# Autodesk Inventor assembly: Baugruppe1
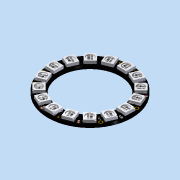
[picture p0: Inventor's stored thumbnail of the model, 180x180]
Saved by Autodesk Inventor 2015 (Build 190159000, 159)
## iProperties
Created: 2015-06-28
Part Number: Baugruppe1
Document SubType Name: Assembly
Designer: M45t3r 0f H4rdc0r3
Author: M45t3r 0f H4rdc0r3
## Documents named in this file (5)
- D:\3D Konstruktion\Neopixelring16x\Dokumentation\Baugruppe1.iam
- D:\3D Konstruktion\Neopixelring16x\Konstruktion\LED-Halter_Ring.ipt
- D:\3D Konstruktion\Neopixelring16x\Importierte Komponenten\WS2812_RGB_LED_updated\WS2812_RGB_LED.ipt
- D:\3D Konstruktion\Neopixelring16x\Importierte Komponenten\CAP0603\CAP0603.ipt
- D:\3D Konstruktion\Neopixelring16x\Importierte Komponenten\RES0603\RES0603_471.ipt
## Components (21 placed, 4 different names)
1. LED-Halter_Ring:1 — Passend:1, Passend:2, Fluchtend:1, Passend:3, Passend:4, Fluchtend:2, Passend:5, Fluchtend:3
2. CAP0603:1 — Passend:2
3. RES0603_471:1 — Fluchtend:1, Passend:3
4. CAP0603:2 — Passend:4, Fluchtend:2
5. CAP0603:3 — Passend:5, Fluchtend:3
6. WS2812_RGB_LED:1 — Passend:1
7. WS2812_RGB_LED:2
8. WS2812_RGB_LED:3
9. WS2812_RGB_LED:4
10. WS2812_RGB_LED:5
11. WS2812_RGB_LED:6
12. WS2812_RGB_LED:7
13. WS2812_RGB_LED:8
14. WS2812_RGB_LED:9
15. WS2812_RGB_LED:10
16. WS2812_RGB_LED:11
17. WS2812_RGB_LED:12
18. WS2812_RGB_LED:13
19. WS2812_RGB_LED:14
20. WS2812_RGB_LED:15
21. WS2812_RGB_LED:16
## Component patterns: (16 elements, first: WS2812_RGB_LED:1)
## Relationships (8: Mate 5, Flush 3)
- Passend:1 [Mate]: LED-Halter_Ring:1 ↔ WS2812_RGB_LED:1
- Passend:2 [Mate]: LED-Halter_Ring:1 ↔ CAP0603:1
- Fluchtend:1 [Flush]: LED-Halter_Ring:1 ↔ RES0603_471:1
- Passend:3 [Mate]: LED-Halter_Ring:1 ↔ RES0603_471:1
- Passend:4 [Mate]: LED-Halter_Ring:1 ↔ CAP0603:2
- Fluchtend:2 [Flush]: LED-Halter_Ring:1 ↔ CAP0603:2
- Passend:5 [Mate]: LED-Halter_Ring:1 ↔ CAP0603:3
- Fluchtend:3 [Flush]: LED-Halter_Ring:1 ↔ CAP0603:3
